# Autodesk Inventor assembly: FinderAssemblyV05
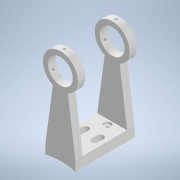
[picture p0: Inventor's stored thumbnail of the model, 180x180]
Saved by Autodesk Inventor 2021 (Build 250183000, 183)
## iProperties
Created: 2020-06-16
Part Number: FinderAssemblyV05
Document SubType Name: Assembly
Designer: robst
Author: robst
## Documents named in this file (3)
- C:\git\CAD-Development\robSteele\ShapeWays\TelescopeProjects\CelestronFinderScope\FinderAssemblyV05.iam
- C:\git\CAD-Development\robSteele\ShapeWays\TelescopeProjects\CelestronFinderScope\finderSupportPartV05.ipt
- C:\git\CAD-Development\robSteele\ShapeWays\TelescopeProjects\CelestronFinderScope\finderMainPartV05.ipt
## Components (2 placed, 2 different names)
1. finderSupportPartV05:1 — Mate:1, Flush:1, Flush:2
2. finderMainPartV05:1 — Mate:1, Flush:1, Flush:2
## Relationships (3: Flush 2, Mate 1)
- Mate:1: finderSupportPartV05:1 ↔ finderMainPartV05:1
- Flush:1: finderSupportPartV05:1 ↔ finderMainPartV05:1
- Flush:2: finderSupportPartV05:1 ↔ finderMainPartV05:1
